# Autodesk Inventor assembly: cellSTORM_v5
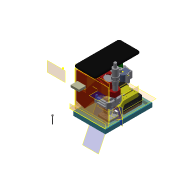
[picture p0: Inventor's stored thumbnail of the model, 180x180]
Saved by Autodesk Inventor 2019.4 (Build 234330000, 330)
## iProperties
Created: 2020-04-25
Part Number: cellSTORM_v5
Document SubType Name: Assembly
Designer: diederichbenedict
Author: diederichbenedict
## Documents named in this file (24)
- C:\Users\diederichbenedict\Dropbox\Dokumente\Promotion\PROJECTS\STORMoChip\GITHUB\CAD\Nanoscopy-on-the-cheap\Workspace\cellSTORM_v5.iam
- C:\Users\diederichbenedict\Dropbox\Dokumente\Promotion\PROJECTS\STORMoChip\GITHUB\CAD\Nanoscopy-on-the-cheap\Workspace\00_XY_stage-CHUO_SEIKI_LD-647-R1.iam
- C:\Users\diederichbenedict\Dropbox\Dokumente\Promotion\PROJECTS\STORMoChip\GITHUB\CAD\Nanoscopy-on-the-cheap\Workspace\cellSTORM_laserbeam.ipt
- C:\Users\diederichbenedict\Dropbox\Dokumente\Promotion\PROJECTS\STORMoChip\GITHUB\CAD\Nanoscopy-on-the-cheap\Workspace\02_Nanoscopy_Chip.ipt
- C:\Users\diederichbenedict\Dropbox\Dokumente\Promotion\PROJECTS\STORMoChip\GITHUB\CAD\Nanoscopy-on-the-cheap\Workspace\00_Ballmagnets_5mm.ipt
- C:\Users\diederichbenedict\Documents\Inventor\Content Center Files\R2019\en-US\DIN 912\DIN 912 - M3 x 0.5 x 25 x 18.ipt
- C:\Users\diederichbenedict\Dropbox\Dokumente\Promotion\PROJECTS\STORMoChip\GITHUB\CAD\Nanoscopy-on-the-cheap\Workspace\00_Huawei_P20.ipt
- C:\Users\diederichbenedict\Dropbox\Dokumente\Promotion\PROJECTS\STORMoChip\GITHUB\CAD\Nanoscopy-on-the-cheap\Workspace\cellSTORM_Base_v0_R1.ipt
- C:\Users\diederichbenedict\Dropbox\Dokumente\Promotion\PROJECTS\STORMoChip\GITHUB\CAD\Nanoscopy-on-the-cheap\Workspace\00_KES400.iam
- C:\Users\diederichbenedict\Dropbox\Dokumente\Promotion\PROJECTS\STORMoChip\GITHUB\CAD\Nanoscopy-on-the-cheap\Workspace\cellSTORM_v5_laserstage.ipt
- C:\Users\diederichbenedict\Dropbox\Dokumente\Promotion\PROJECTS\STORMoChip\GITHUB\CAD\Nanoscopy-on-the-cheap\Workspace\cellSTORM_v5_cellphonestage.ipt
- C:\Users\diederichbenedict\Dropbox\Dokumente\Promotion\PROJECTS\STORMoChip\GITHUB\CAD\Nanoscopy-on-the-cheap\Workspace\cellSTORM_v5_microsocpe.iam
- C:\Users\diederichbenedict\Dropbox\Dokumente\Promotion\PROJECTS\STORMoChip\GITHUB\CAD\Nanoscopy-on-the-cheap\Workspace\cellSTORM_v5_microscope_cover.ipt
- C:\Users\diederichbenedict\Dropbox\Dokumente\Promotion\PROJECTS\STORMoChip\GITHUB\CAD\Nanoscopy-on-the-cheap\Workspace\00_Stepper_Motor_28BYJ-48.0013.ipt
- C:\Users\diederichbenedict\Dropbox\Dokumente\Promotion\PROJECTS\STORMoChip\GITHUB\CAD\Nanoscopy-on-the-cheap\Workspace\cellSTORM_v5_focusmotormount.ipt
- C:\Users\diederichbenedict\Dropbox\Dokumente\Promotion\PROJECTS\STORMoChip\GITHUB\CAD\Nanoscopy-on-the-cheap\Workspace\BD-DRIVE_PULLEY.ipt
- C:\Users\diederichbenedict\Dropbox\Dokumente\Promotion\PROJECTS\STORMoChip\GITHUB\CAD\Nanoscopy-on-the-cheap\Workspace\cellSTORM_focusmotor_pulley.ipt
- C:\Users\diederichbenedict\Dropbox\Dokumente\Promotion\PROJECTS\STORMoChip\GITHUB\CAD\Nanoscopy-on-the-cheap\Workspace\00_chip_01_old.ipt
- C:\Users\diederichbenedict\Dropbox\Dokumente\Promotion\PROJECTS\STORMoChip\GITHUB\CAD\Nanoscopy-on-the-cheap\Workspace\cellSTORM_v5_chiptray_old_0.ipt
- C:\Users\diederichbenedict\Dropbox\Dokumente\Promotion\PROJECTS\STORMoChip\GITHUB\CAD\Nanoscopy-on-the-cheap\Workspace\cellSTORM_v5_chiptry_clamp.ipt
- C:\Users\diederichbenedict\Dropbox\Dokumente\Promotion\PROJECTS\STORMoChip\GITHUB\CAD\Nanoscopy-on-the-cheap\Workspace\00_Laser_532nm_200mw.ipt
- C:\Users\diederichbenedict\Dropbox\Dokumente\Promotion\PROJECTS\STORMoChip\GITHUB\CAD\Nanoscopy-on-the-cheap\Workspace\cellSTORM_v5_cellphonespacer.ipt
- C:\Users\diederichbenedict\Documents\Inventor\Content Center Files\R2019\en-US\DIN 912\DIN 912 - M3 x 0.5 x 20 x 18.75.ipt
- C:\Users\diederichbenedict\Documents\Inventor\Content Center Files\R2019\en-US\DIN 912\DIN 912 - M4 x 0.7 x 10 x 8.25.ipt
## Components (40 placed, 23 different names)
1. 00_XY_stage-CHUO_SEIKI_LD-647-R1:1 [sub-assembly] — Insert:1, Angle:1, Insert:6, Angle:5, Flush:10, Flush:11
2. cellSTORM_laserbeam:1 — Insert:3, Insert:7, Insert:16, Mate:27
3. 02_Nanoscopy_Chip:1 — Insert:3, Angle:2, Mate:11
4. 00_Ballmagnets_5mm:1
5. DIN 912 - replaced by DIN EN ISO 4762 M3 x 25:1 — Insert:4
6. 00_Ballmagnets_5mm:2
7. DIN 912 - replaced by DIN EN ISO 4762 M3 x 25:2 — Insert:13
8. 00_Ballmagnets_5mm:3
9. DIN 912 - replaced by DIN EN ISO 4762 M3 x 25:3 — Insert:14
10. cellSTORM_Base_v0_R1:1 — Insert:1, Angle:1, Angle:2, Insert:4, Insert:13, Insert:14, Flush:23, Insert:20, Insert:21, Insert:22, Insert:23
11. 00_XY_stage-CHUO_SEIKI_LD-647-R1:2 [sub-assembly] — Insert:6, Angle:5, Flush:12, Flush:13, Flush:32
12. 00_KES400:1 [sub-assembly] — Insert:7, Mate:27, Mate:28
13. cellSTORM_v5_laserstage:1 — Flush:10, Flush:11, Insert:19, Mate:29
14. cellSTORM_v5_cellphonestage:1 — Flush:12, Flush:13, Mate:10, Flush:14, Flush:17, Flush:18, Flush:19, Mate:24
15. cellSTORM_v5_microsocpe:1 [sub-assembly] — Mate:10, Mate:11, Flush:14, Flush:15, Flush:16, Mate:18, Mate:19, Mate:23, Insert:17
16. cellSTORM_v5_microscope_cover:1 — Flush:15, Flush:16
17. 00_Stepper_Motor_28BYJ-48.0013:1 — Mate:18, Mate:19, Flush:17, Flush:20, Insert:15, Insert:27, Insert:28
18. cellSTORM_v5_focusmotormount:1 — Flush:18, Flush:19, Flush:20, Flush:31, Insert:24, Insert:25, Insert:26
19. BD-DRIVE_PULLEY:1 — Insert:15
20. 00_Huawei_P20:1 — Mate:23, Mate:24
21. 00_chip_01_old:1 — Flush:22, Insert:16
22. cellSTORM_v5_chiptray_old_0:1 — Flush:22, Flush:23, Flush:24, Flush:25
23. cellSTORM_v5_chiptry_clamp:1 — Flush:24, Flush:25
24. 00_Laser_532nm_200mw:1 — Mate:28
25. cellSTORM_v5_cellphonespacer:1 — Flush:31, Flush:32
26. cellSTORM_focusmotor_pulley:1 — Insert:17
27. DIN 912 - replaced by DIN EN ISO 4762 M3 x 25:4
28. DIN 912 - replaced by DIN EN ISO 4762 M3 x 20:1 — Insert:28
29. DIN 912 - replaced by DIN EN ISO 4762 M3 x 20:2 — Mate:29
30. DIN 912 - replaced by DIN EN ISO 4762 M3 x 20:4 — Insert:19
31. DIN 912 - replaced by DIN EN ISO 4762 M3 x 20:5 — Insert:27
32. DIN 912 - replaced by DIN EN ISO 4762 M3 x 20:6
33. DIN 912 - replaced by DIN EN ISO 4762 M4 x 10:1 — Insert:22
34. DIN 912 - replaced by DIN EN ISO 4762 M4 x 10:2 — Insert:24
35. DIN 912 - replaced by DIN EN ISO 4762 M4 x 10:3 — Insert:25
36. DIN 912 - replaced by DIN EN ISO 4762 M4 x 10:4 — Insert:23
37. DIN 912 - replaced by DIN EN ISO 4762 M4 x 10:5 — Insert:26
38. DIN 912 - replaced by DIN EN ISO 4762 M4 x 10:6 — Insert:21
39. DIN 912 - replaced by DIN EN ISO 4762 M4 x 10:7 — Insert:20
40. DIN 912 - replaced by DIN EN ISO 4762 M3 x 20:7
## Relationships (52: Insert 20, Flush 17, Mate 12, Angle 3)
- [Mate]: 00_Ballmagnets_5mm:1 ↔ DIN 912 - replaced by DIN EN ISO 4762 M3 x 25:1
- [Mate]: 00_Ballmagnets_5mm:2 ↔ DIN 912 - replaced by DIN EN ISO 4762 M3 x 25:2
- [Mate]: 00_Ballmagnets_5mm:3 ↔ DIN 912 - replaced by DIN EN ISO 4762 M3 x 25:3
- Insert:1: 00_XY_stage-CHUO_SEIKI_LD-647-R1:1 ↔ cellSTORM_Base_v0_R1:1
- Angle:1 (90 deg): 00_XY_stage-CHUO_SEIKI_LD-647-R1:1 ↔ cellSTORM_Base_v0_R1:1
- Insert:3 (5 mm): cellSTORM_laserbeam:1 ↔ 02_Nanoscopy_Chip:1
- Angle:2 (180 deg): 02_Nanoscopy_Chip:1 ↔ cellSTORM_Base_v0_R1:1
- Insert:4 (-15 mm): DIN 912 - replaced by DIN EN ISO 4762 M3 x 25:1 ↔ cellSTORM_Base_v0_R1:1
- Insert:6 (6 mm): 00_XY_stage-CHUO_SEIKI_LD-647-R1:1 ↔ 00_XY_stage-CHUO_SEIKI_LD-647-R1:2
- Angle:5 (180 deg): 00_XY_stage-CHUO_SEIKI_LD-647-R1:1 ↔ 00_XY_stage-CHUO_SEIKI_LD-647-R1:2
- Insert:7: cellSTORM_laserbeam:1 ↔ 00_KES400:1
- Insert:13 (-15 mm): DIN 912 - replaced by DIN EN ISO 4762 M3 x 25:2 ↔ cellSTORM_Base_v0_R1:1
- Insert:14 (-15 mm): DIN 912 - replaced by DIN EN ISO 4762 M3 x 25:3 ↔ cellSTORM_Base_v0_R1:1
- Flush:10: 00_XY_stage-CHUO_SEIKI_LD-647-R1:1 ↔ cellSTORM_v5_laserstage:1
- Flush:11: 00_XY_stage-CHUO_SEIKI_LD-647-R1:1 ↔ cellSTORM_v5_laserstage:1
- Flush:12: 00_XY_stage-CHUO_SEIKI_LD-647-R1:2 ↔ cellSTORM_v5_cellphonestage:1
- Flush:13: 00_XY_stage-CHUO_SEIKI_LD-647-R1:2 ↔ cellSTORM_v5_cellphonestage:1
- Mate:10: cellSTORM_v5_cellphonestage:1 ↔ cellSTORM_v5_microsocpe:1
- Mate:11: 02_Nanoscopy_Chip:1 ↔ cellSTORM_v5_microsocpe:1
- Flush:14: cellSTORM_v5_cellphonestage:1 ↔ cellSTORM_v5_microsocpe:1
- Flush:15: cellSTORM_v5_microsocpe:1 ↔ cellSTORM_v5_microscope_cover:1
- Flush:16: cellSTORM_v5_microsocpe:1 ↔ cellSTORM_v5_microscope_cover:1
- Mate:18 (10 mm): cellSTORM_v5_microsocpe:1 ↔ 00_Stepper_Motor_28BYJ-48.0013:1
- Mate:19 (35 mm): cellSTORM_v5_microsocpe:1 ↔ 00_Stepper_Motor_28BYJ-48.0013:1
- Flush:17 (-40 mm): cellSTORM_v5_cellphonestage:1 ↔ 00_Stepper_Motor_28BYJ-48.0013:1
- Flush:18: cellSTORM_v5_cellphonestage:1 ↔ cellSTORM_v5_focusmotormount:1
- Flush:19: cellSTORM_v5_cellphonestage:1 ↔ cellSTORM_v5_focusmotormount:1
- Flush:20: 00_Stepper_Motor_28BYJ-48.0013:1 ↔ cellSTORM_v5_focusmotormount:1
- Insert:15: 00_Stepper_Motor_28BYJ-48.0013:1 ↔ BD-DRIVE_PULLEY:1
- Mate:23: cellSTORM_v5_microsocpe:1 ↔ 00_Huawei_P20:1
- Mate:24: cellSTORM_v5_cellphonestage:1 ↔ 00_Huawei_P20:1
- Flush:22: 00_chip_01_old:1 ↔ cellSTORM_v5_chiptray_old_0:1
- Flush:23 (10 mm): cellSTORM_Base_v0_R1:1 ↔ cellSTORM_v5_chiptray_old_0:1
- Insert:16: cellSTORM_laserbeam:1 ↔ 00_chip_01_old:1
- Flush:24: cellSTORM_v5_chiptray_old_0:1 ↔ cellSTORM_v5_chiptry_clamp:1
- Flush:25: cellSTORM_v5_chiptray_old_0:1 ↔ cellSTORM_v5_chiptry_clamp:1
- Mate:27: cellSTORM_laserbeam:1 ↔ 00_KES400:1
- Mate:28: 00_KES400:1 ↔ 00_Laser_532nm_200mw:1
- Flush:31: cellSTORM_v5_focusmotormount:1 ↔ cellSTORM_v5_cellphonespacer:1
- Flush:32: 00_XY_stage-CHUO_SEIKI_LD-647-R1:2 ↔ cellSTORM_v5_cellphonespacer:1
- Insert:17 (23 mm): cellSTORM_v5_microsocpe:1 ↔ cellSTORM_focusmotor_pulley:1
- Insert:19: cellSTORM_v5_laserstage:1 ↔ DIN 912 - replaced by DIN EN ISO 4762 M3 x 20:4
- Mate:29: cellSTORM_v5_laserstage:1 ↔ DIN 912 - replaced by DIN EN ISO 4762 M3 x 20:2
- Insert:20: cellSTORM_Base_v0_R1:1 ↔ DIN 912 - replaced by DIN EN ISO 4762 M4 x 10:7
- Insert:21: cellSTORM_Base_v0_R1:1 ↔ DIN 912 - replaced by DIN EN ISO 4762 M4 x 10:6
- Insert:22: cellSTORM_Base_v0_R1:1 ↔ DIN 912 - replaced by DIN EN ISO 4762 M4 x 10:1
- Insert:23: cellSTORM_Base_v0_R1:1 ↔ DIN 912 - replaced by DIN EN ISO 4762 M4 x 10:4
- Insert:24: cellSTORM_v5_focusmotormount:1 ↔ DIN 912 - replaced by DIN EN ISO 4762 M4 x 10:2
- Insert:25: cellSTORM_v5_focusmotormount:1 ↔ DIN 912 - replaced by DIN EN ISO 4762 M4 x 10:3
- Insert:26: cellSTORM_v5_focusmotormount:1 ↔ DIN 912 - replaced by DIN EN ISO 4762 M4 x 10:5
- Insert:27: 00_Stepper_Motor_28BYJ-48.0013:1 ↔ DIN 912 - replaced by DIN EN ISO 4762 M3 x 20:5
- Insert:28: 00_Stepper_Motor_28BYJ-48.0013:1 ↔ DIN 912 - replaced by DIN EN ISO 4762 M3 x 20:1
## Named parameters: d2_d162 = 0 mm, d3_d162 = 0 mm
